# Autodesk Inventor assembly: aluminumFramePowerCellLauncherV01
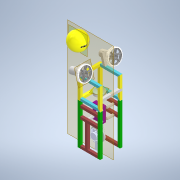
[picture p0: Inventor's stored thumbnail of the model, 180x180]
Saved by Autodesk Inventor 2020.2 (Build 242310000, 310)
## iProperties
Created: 2020-01-17
Part Number: aluminumFramePowerCellLauncherV01
Document SubType Name: Assembly
Designer: robst
Author: robst
## Documents named in this file (17)
- C:\git\CAD-Development\robSteele\2020BallTriggerMechanism\aluminumFramePowerCellLauncherV01.iam
- C:\git\CAD-Development\robSteele\2020BallTriggerMechanism\8-inchAluminumTubing.ipt
- C:\git\CAD-Development\robSteele\2020BallTriggerMechanism\motorBracket01.ipt
- C:\git\CAD-Development\robSteele\2020BallTriggerMechanism\6inchMiniCimShooter.iam
- C:\git\CAD-Development\robSteele\2020BallTriggerMechanism\9_250-inchAluminumTubingWith45DegreeCuts.ipt
- C:\git\CAD-Development\robSteele\2020BallTriggerMechanism\1892-YEL.ipt
- C:\git\CAD-Development\robSteele\2020BallTriggerMechanism\8_250-inchAluminumTubingWithOne45DegreeCut.ipt
- C:\git\CAD-Development\robSteele\2020BallTriggerMechanism\pistonMechanism.iam
- C:\git\CAD-Development\robSteele\2020BallTriggerMechanism\7_250-inchAluminumTubing.ipt
- C:\git\CAD-Development\robSteele\2020BallTriggerMechanism\17-inchAluminumTubing.ipt
- C:\git\CAD-Development\robSteele\2020BallTriggerMechanism\2_875-spacers.ipt
- C:\git\CAD-Development\robSteele\2020BallTriggerMechanism\9_500-inchAluminumTubing.ipt
- C:\git\CAD-Development\robSteele\2020BallTriggerMechanism\motorBracket01_MIR2.ipt
- C:\git\CAD-Development\robSteele\2020BallTriggerMechanism\6inchMiniCimShooter_MIR2.iam
- C:\git\CAD-Development\robSteele\2020BallTriggerMechanism\17-inchAluminumTubing_MIR.ipt
- C:\git\CAD-Development\robSteele\2020BallTriggerMechanism\7_250-inchAluminumTubing_MIR.ipt
- C:\git\CAD-Development\robSteele\2020BallTriggerMechanism\2_875-spacers_MIR.ipt
## Components (37 placed, 16 different names)
1. 9_250-inchAluminumTubingWith45DegreeCuts:1 — Mate:1, Flush:1, Mate:4, Mate:9, Mate:10, Flush:13, Flush:15, Mate:29
2. 9_250-inchAluminumTubingWith45DegreeCuts:2 — Mate:1, Flush:1, Mate:2, Mate:3, Flush:2, Mate:4, Flush:5, Flush:14, Mate:25
3. 9_250-inchAluminumTubingWith45DegreeCuts:3 — Mate:2, Mate:3, Flush:2, Mate:5, Flush:3, Mate:6, Mate:7, Flush:4, Mate:8, Flush:6, Mate:20
4. 9_250-inchAluminumTubingWith45DegreeCuts:4 — Mate:5, Flush:3, Mate:6, Flush:7, Flush:12, Flush:25, Flush:31, Flush:32
5. 8_250-inchAluminumTubingWithOne45DegreeCut:1 — Mate:7, Flush:4, Flush:5, Mate:11, Mate:12, Flush:16
6. 8_250-inchAluminumTubingWithOne45DegreeCut:2 — Mate:8, Flush:6, Flush:7, Mate:13, Mate:14, Flush:17, Flush:19, Mate:16, Flush:20
7. 8_250-inchAluminumTubingWithOne45DegreeCut:3 — Mate:9, Flush:12, Flush:13, Mate:30, Flush:33, Mate:33
8. 8_250-inchAluminumTubingWithOne45DegreeCut:4 — Mate:10, Flush:14, Flush:15
9. 9_250-inchAluminumTubingWith45DegreeCuts:5 — Mate:13, Mate:14, Flush:17, Mate:15, Flush:18, Mate:23, Flush:34
10. 9_250-inchAluminumTubingWith45DegreeCuts:6 — Mate:11, Mate:12, Flush:16, Mate:24
11. 8-inchAluminumTubing:1 — Mate:15, Flush:18, Flush:19
12. motorBracket01:1 — Mate:16, Flush:20, Mate:17, Flush:21, Flush:22, Mate:20
13. 6inchMiniCimShooter:1 [sub-assembly] — Mate:17, Flush:21, Flush:22
14. 1892-YEL:1 — Mate:19, Mate:21
15. pistonMechanism:1 [sub-assembly] — Insert:1, Insert:2, Insert:3, Insert:4
16. 17-inchAluminumTubing:1 — Mate:29, Flush:31, Flush:32, Mate:31, Flush:35, Flush:36, Mate:32, Flush:39, Mate:34, Flush:40, Mate:37
17. 17-inchAluminumTubing:2 — Mate:30, Flush:33, Flush:34
18. 7_250-inchAluminumTubing:2 — Mate:31, Flush:35, Flush:36, Mate:36, Flush:41
19. 7_250-inchAluminumTubing:3 — Mate:32, Flush:39, Mate:33, Mate:35
20. 7_250-inchAluminumTubing:4 — Mate:34, Flush:40, Mate:35
21. 2_875-spacers:1 — Insert:1
22. 2_875-spacers:2 — Insert:2
23. 2_875-spacers:3 — Insert:3
24. 2_875-spacers:4 — Insert:4
25. 9_500-inchAluminumTubing:1 — Mate:36, Flush:41, Mate:37
26. motorBracket01_MIR2:1 — Flush:42, Flush:43, Mate:38
27. 6inchMiniCimShooter_MIR2:1 [sub-assembly] — Flush:42, Flush:43, Mate:38
28. 17-inchAluminumTubing_MIR:1 — Flush:44, Flush:45, Mate:39, Flush:46, Mate:40, Flush:47, Mate:42
29. 17-inchAluminumTubing_MIR:2
30. 7_250-inchAluminumTubing_MIR:1 — Flush:44, Flush:45, Mate:39
31. 7_250-inchAluminumTubing_MIR:2 — Flush:46, Mate:40, Mate:41
32. 7_250-inchAluminumTubing_MIR:3 — Mate:41, Flush:47, Mate:42
33. 2_875-spacers_MIR:1
34. 2_875-spacers_MIR:2
35. 2_875-spacers_MIR:3
36. 2_875-spacers_MIR:4
37. 1892-YEL:2 — Mate:43
## Relationships (76: Mate 38, Flush 34, Insert 4)
- Mate:1: 9_250-inchAluminumTubingWith45DegreeCuts:1 ↔ 9_250-inchAluminumTubingWith45DegreeCuts:2
- Flush:1: 9_250-inchAluminumTubingWith45DegreeCuts:1 ↔ 9_250-inchAluminumTubingWith45DegreeCuts:2
- Mate:2: 9_250-inchAluminumTubingWith45DegreeCuts:2 ↔ 9_250-inchAluminumTubingWith45DegreeCuts:3
- Mate:3: 9_250-inchAluminumTubingWith45DegreeCuts:2 ↔ 9_250-inchAluminumTubingWith45DegreeCuts:3
- Flush:2: 9_250-inchAluminumTubingWith45DegreeCuts:2 ↔ 9_250-inchAluminumTubingWith45DegreeCuts:3
- Mate:4: 9_250-inchAluminumTubingWith45DegreeCuts:1 ↔ 9_250-inchAluminumTubingWith45DegreeCuts:2
- Mate:5: 9_250-inchAluminumTubingWith45DegreeCuts:3 ↔ 9_250-inchAluminumTubingWith45DegreeCuts:4
- Flush:3: 9_250-inchAluminumTubingWith45DegreeCuts:3 ↔ 9_250-inchAluminumTubingWith45DegreeCuts:4
- Mate:6: 9_250-inchAluminumTubingWith45DegreeCuts:3 ↔ 9_250-inchAluminumTubingWith45DegreeCuts:4
- Mate:7: 9_250-inchAluminumTubingWith45DegreeCuts:3 ↔ 8_250-inchAluminumTubingWithOne45DegreeCut:1
- Flush:4: 9_250-inchAluminumTubingWith45DegreeCuts:3 ↔ 8_250-inchAluminumTubingWithOne45DegreeCut:1
- Flush:5: 9_250-inchAluminumTubingWith45DegreeCuts:2 ↔ 8_250-inchAluminumTubingWithOne45DegreeCut:1
- Mate:8: 9_250-inchAluminumTubingWith45DegreeCuts:3 ↔ 8_250-inchAluminumTubingWithOne45DegreeCut:2
- Flush:6: 9_250-inchAluminumTubingWith45DegreeCuts:3 ↔ 8_250-inchAluminumTubingWithOne45DegreeCut:2
- Flush:7: 9_250-inchAluminumTubingWith45DegreeCuts:4 ↔ 8_250-inchAluminumTubingWithOne45DegreeCut:2
- Mate:9: 9_250-inchAluminumTubingWith45DegreeCuts:1 ↔ 8_250-inchAluminumTubingWithOne45DegreeCut:3
- Mate:10: 9_250-inchAluminumTubingWith45DegreeCuts:1 ↔ 8_250-inchAluminumTubingWithOne45DegreeCut:4
- Flush:12: 9_250-inchAluminumTubingWith45DegreeCuts:4 ↔ 8_250-inchAluminumTubingWithOne45DegreeCut:3
- Flush:13: 9_250-inchAluminumTubingWith45DegreeCuts:1 ↔ 8_250-inchAluminumTubingWithOne45DegreeCut:3
- Flush:14: 9_250-inchAluminumTubingWith45DegreeCuts:2 ↔ 8_250-inchAluminumTubingWithOne45DegreeCut:4
- Flush:15: 9_250-inchAluminumTubingWith45DegreeCuts:1 ↔ 8_250-inchAluminumTubingWithOne45DegreeCut:4
- Mate:11: 8_250-inchAluminumTubingWithOne45DegreeCut:1 ↔ 9_250-inchAluminumTubingWith45DegreeCuts:6
- Mate:12: 8_250-inchAluminumTubingWithOne45DegreeCut:1 ↔ 9_250-inchAluminumTubingWith45DegreeCuts:6
- Flush:16: 8_250-inchAluminumTubingWithOne45DegreeCut:1 ↔ 9_250-inchAluminumTubingWith45DegreeCuts:6
- Mate:13: 8_250-inchAluminumTubingWithOne45DegreeCut:2 ↔ 9_250-inchAluminumTubingWith45DegreeCuts:5
- Mate:14: 8_250-inchAluminumTubingWithOne45DegreeCut:2 ↔ 9_250-inchAluminumTubingWith45DegreeCuts:5
- Flush:17: 8_250-inchAluminumTubingWithOne45DegreeCut:2 ↔ 9_250-inchAluminumTubingWith45DegreeCuts:5
- Mate:15: 9_250-inchAluminumTubingWith45DegreeCuts:5 ↔ 8-inchAluminumTubing:1
- Flush:18: 9_250-inchAluminumTubingWith45DegreeCuts:5 ↔ 8-inchAluminumTubing:1
- Flush:19 (-127 mm): 8_250-inchAluminumTubingWithOne45DegreeCut:2 ↔ 8-inchAluminumTubing:1
- Mate:16: 8_250-inchAluminumTubingWithOne45DegreeCut:2 ↔ motorBracket01:1
- Flush:20: 8_250-inchAluminumTubingWithOne45DegreeCut:2 ↔ motorBracket01:1
- Mate:17: motorBracket01:1 ↔ 6inchMiniCimShooter:1
- Flush:21: motorBracket01:1 ↔ 6inchMiniCimShooter:1
- Flush:22: motorBracket01:1 ↔ 6inchMiniCimShooter:1
- Mate:19: 1892-YEL:1
- Mate:20 (-50.8 mm): 9_250-inchAluminumTubingWith45DegreeCuts:3 ↔ motorBracket01:1
- Flush:25 (92.075 mm): 9_250-inchAluminumTubingWith45DegreeCuts:4
- Mate:21: 1892-YEL:1
- Mate:23: 9_250-inchAluminumTubingWith45DegreeCuts:5
- Mate:24: 9_250-inchAluminumTubingWith45DegreeCuts:6
- Mate:25: 9_250-inchAluminumTubingWith45DegreeCuts:2
- Mate:29: 9_250-inchAluminumTubingWith45DegreeCuts:1 ↔ 17-inchAluminumTubing:1
- Flush:31: 9_250-inchAluminumTubingWith45DegreeCuts:4 ↔ 17-inchAluminumTubing:1
- Flush:32: 9_250-inchAluminumTubingWith45DegreeCuts:4 ↔ 17-inchAluminumTubing:1
- Mate:30: 8_250-inchAluminumTubingWithOne45DegreeCut:3 ↔ 17-inchAluminumTubing:2
- Flush:33: 8_250-inchAluminumTubingWithOne45DegreeCut:3 ↔ 17-inchAluminumTubing:2
- Flush:34: 9_250-inchAluminumTubingWith45DegreeCuts:5 ↔ 17-inchAluminumTubing:2
- Mate:31: 17-inchAluminumTubing:1 ↔ 7_250-inchAluminumTubing:2
- Flush:35: 17-inchAluminumTubing:1 ↔ 7_250-inchAluminumTubing:2
- Flush:36: 17-inchAluminumTubing:1 ↔ 7_250-inchAluminumTubing:2
- Mate:32: 17-inchAluminumTubing:1 ↔ 7_250-inchAluminumTubing:3
- Flush:39: 17-inchAluminumTubing:1 ↔ 7_250-inchAluminumTubing:3
- Mate:33 (38.1 mm): 8_250-inchAluminumTubingWithOne45DegreeCut:3 ↔ 7_250-inchAluminumTubing:3
- Mate:34: 17-inchAluminumTubing:1 ↔ 7_250-inchAluminumTubing:4
- Flush:40: 17-inchAluminumTubing:1 ↔ 7_250-inchAluminumTubing:4
- Mate:35 (76.2 mm): 7_250-inchAluminumTubing:3 ↔ 7_250-inchAluminumTubing:4
- Insert:1: pistonMechanism:1 ↔ 2_875-spacers:1
- Insert:2: pistonMechanism:1 ↔ 2_875-spacers:2
- Insert:3: pistonMechanism:1 ↔ 2_875-spacers:3
- Insert:4: pistonMechanism:1 ↔ 2_875-spacers:4
- Mate:36: 7_250-inchAluminumTubing:2 ↔ 9_500-inchAluminumTubing:1
- Flush:41: 7_250-inchAluminumTubing:2 ↔ 9_500-inchAluminumTubing:1
- Mate:37 (50.8 mm): 17-inchAluminumTubing:1 ↔ 9_500-inchAluminumTubing:1
- Flush:42: motorBracket01_MIR2:1 ↔ 6inchMiniCimShooter_MIR2:1
- Flush:43: motorBracket01_MIR2:1 ↔ 6inchMiniCimShooter_MIR2:1
- Mate:38: motorBracket01_MIR2:1 ↔ 6inchMiniCimShooter_MIR2:1
- Flush:44: 17-inchAluminumTubing_MIR:1 ↔ 7_250-inchAluminumTubing_MIR:1
- Flush:45: 17-inchAluminumTubing_MIR:1 ↔ 7_250-inchAluminumTubing_MIR:1
- Mate:39: 17-inchAluminumTubing_MIR:1 ↔ 7_250-inchAluminumTubing_MIR:1
- Flush:46: 17-inchAluminumTubing_MIR:1 ↔ 7_250-inchAluminumTubing_MIR:2
- Mate:40: 17-inchAluminumTubing_MIR:1 ↔ 7_250-inchAluminumTubing_MIR:2
- Mate:41 (76.2 mm): 7_250-inchAluminumTubing_MIR:2 ↔ 7_250-inchAluminumTubing_MIR:3
- Flush:47: 17-inchAluminumTubing_MIR:1 ↔ 7_250-inchAluminumTubing_MIR:3
- Mate:42: 17-inchAluminumTubing_MIR:1 ↔ 7_250-inchAluminumTubing_MIR:3
- Mate:43: 1892-YEL:2
